# Autodesk Inventor assembly: AA00001098209
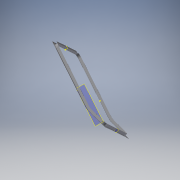
[picture p0: Inventor's stored thumbnail of the model, 180x180]
Saved by Autodesk Inventor 2017 (Build 210142000, 142)
## iProperties
Created: 2019-04-08
Part Number: AA00001098209
Document SubType Name: Assembly
Designer: Phs
Author: Phs
## Documents named in this file (11)
- C:\Users\Phs\Documents\Inventor\Eriyeti Murena\AA00001098209.iam
- C:\Users\Phs\Documents\Inventor\Eriyeti Murena\AAD0001344795.ipt
- C:\Users\Phs\Documents\Inventor\Eriyeti Murena\DTD0000254432.ipt
- C:\Users\Phs\Documents\Inventor\Eriyeti Murena\DTD0000254439.ipt
- C:\Users\Phs\Documents\Inventor\Eriyeti Murena\AAD0001098233.ipt
- C:\Users\Phs\Documents\Inventor\Eriyeti Murena\DTD0000254398.ipt
- C:\Users\Phs\Documents\Inventor\Eriyeti Murena\AAD0001344795_MIR.ipt
- C:\Users\Phs\Documents\Inventor\Eriyeti Murena\DTD0000254439_MIR.ipt
- C:\Users\Phs\Documents\Inventor\Eriyeti Murena\DTD0000254432_MIR.ipt
- C:\Users\Phs\Documents\Inventor\Eriyeti Murena\AAD0001098233_MIR.ipt
- C:\Users\Phs\Documents\Inventor\Eriyeti Murena\DTD0000254419.ipt
## Components (10 placed, 10 different names)
1. AAD0001344795:1 — Mate:2, Flush:1, Flush:2, Flush:3, Flush:4, Flush:5, Mate:8
2. DTD0000254439:1 — Mate:2, Flush:1, Flush:2, Mate:3, Flush:6, Flush:7
3. DTD0000254432:1 — Flush:3, Flush:4, Flush:5
4. AAD0001098233:1 — Mate:3, Flush:6, Flush:7, Mate:4, Flush:8, Flush:9
5. DTD0000254398:1 — Mate:4, Flush:8, Flush:9, Flush:19, Mate:10, Flush:20, Flush:21
6. AAD0001344795_MIR:1 — Flush:10, Flush:11, Mate:5, Flush:12, Flush:13, Flush:14, Mate:9
7. DTD0000254439_MIR:1 — Flush:10, Flush:11, Mate:5, Flush:15, Flush:16, Mate:6
8. DTD0000254432_MIR:1 — Flush:12, Flush:13, Flush:14
9. AAD0001098233_MIR:1 — Flush:15, Flush:16, Mate:6, Mate:10, Flush:20, Flush:21
10. DTD0000254419:1 — Mate:8, Flush:19, Mate:9
## Relationships (27: Flush 19, Mate 8)
- Mate:2: AAD0001344795:1 ↔ DTD0000254439:1
- Flush:1: AAD0001344795:1 ↔ DTD0000254439:1
- Flush:2: AAD0001344795:1 ↔ DTD0000254439:1
- Flush:3: AAD0001344795:1 ↔ DTD0000254432:1
- Flush:4: AAD0001344795:1 ↔ DTD0000254432:1
- Flush:5: AAD0001344795:1 ↔ DTD0000254432:1
- Mate:3: DTD0000254439:1 ↔ AAD0001098233:1
- Flush:6: DTD0000254439:1 ↔ AAD0001098233:1
- Flush:7: DTD0000254439:1 ↔ AAD0001098233:1
- Mate:4: AAD0001098233:1 ↔ DTD0000254398:1
- Flush:8: AAD0001098233:1 ↔ DTD0000254398:1
- Flush:9: AAD0001098233:1 ↔ DTD0000254398:1
- Flush:10: AAD0001344795_MIR:1 ↔ DTD0000254439_MIR:1
- Flush:11: AAD0001344795_MIR:1 ↔ DTD0000254439_MIR:1
- Mate:5: AAD0001344795_MIR:1 ↔ DTD0000254439_MIR:1
- Flush:12: AAD0001344795_MIR:1 ↔ DTD0000254432_MIR:1
- Flush:13: AAD0001344795_MIR:1 ↔ DTD0000254432_MIR:1
- Flush:14: AAD0001344795_MIR:1 ↔ DTD0000254432_MIR:1
- Flush:15: DTD0000254439_MIR:1 ↔ AAD0001098233_MIR:1
- Flush:16: DTD0000254439_MIR:1 ↔ AAD0001098233_MIR:1
- Mate:6: DTD0000254439_MIR:1 ↔ AAD0001098233_MIR:1
- Mate:8: AAD0001344795:1 ↔ DTD0000254419:1
- Flush:19: DTD0000254398:1 ↔ DTD0000254419:1
- Mate:9: AAD0001344795_MIR:1 ↔ DTD0000254419:1
- Mate:10: DTD0000254398:1 ↔ AAD0001098233_MIR:1
- Flush:20: DTD0000254398:1 ↔ AAD0001098233_MIR:1
- Flush:21: DTD0000254398:1 ↔ AAD0001098233_MIR:1
